# Autodesk Inventor assembly: Vex Traction Wheel 6x1
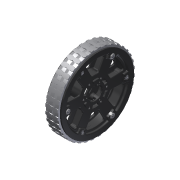
[picture p0: Inventor's stored thumbnail of the model, 180x180]
Saved by Autodesk Inventor 2013 (Build 170138000, 138)
## iProperties
Created: 2012-12-09
Part Number: Vex Traction Wheel 6x1
Document SubType Name: Assembly
Designer: Nemo
Author: Nemo
## Documents named in this file (6)
- H:\Nemo\Documents\Robotics\COTS Parts\Wheels\VexPro Traction Wheels\Vex Traction Wheel 6x1.iam
- H:\Nemo\Documents\Robotics\COTS Parts\Wheels\VexPro Traction Wheels\Components\Traction Wheel Body 6in.ipt
- H:\Nemo\Documents\Robotics\COTS Parts\Fasteners\Hex Standoff 8-32 x750.ipt
- H:\Nemo\Documents\Robotics\COTS Parts\Fasteners\8-32 locknut.ipt
- H:\Nemo\Documents\Robotics\COTS Parts\Fasteners\8-32 BHCS x1250.ipt
- H:\Nemo\Documents\Robotics\COTS Parts\Wheels\VexPro Traction Wheels\Components\6 in Traction Tire.iam
## Components (22 placed, 5 different names)
1. Traction Wheel Body 6in:1 — Mate:1, Flush:1, Mate:2, Angle:1, Insert:1, Insert:2, Angle:2, Insert:3, Mate:5, Mate:8
2. Traction Wheel Body 6in:2 — Mate:3, Mate:4, Mate:5, Insert:4, Angle:3, Insert:5
3. 6 in Traction Tire:1 [sub-assembly] — Mate:6, Mate:7, Mate:8, Mate:11
4. 6 in Traction Tire:2 [sub-assembly] — Mate:9, Mate:10, Mate:11
5. Hex Standoff 8-32 x750:1 — Angle:1, Insert:1
6. Hex Standoff 8-32 x750:2
7. Hex Standoff 8-32 x750:3
8. Hex Standoff 8-32 x750:4
9. Hex Standoff 8-32 x750:5
10. Hex Standoff 8-32 x750:6
11. 8-32 BHCS x1250:2 — Insert:4
12. 8-32 locknut:2 — Angle:3, Insert:5
13. 8-32 BHCS x1250:1 — Insert:3
14. 8-32 locknut:1 — Insert:2, Angle:2
15. 8-32 BHCS x1250:3
16. 8-32 locknut:3
17. 8-32 BHCS x1250:4
18. 8-32 locknut:4
19. 8-32 BHCS x1250:5
20. 8-32 locknut:5
21. 8-32 BHCS x1250:6
22. 8-32 locknut:6
## Component patterns: (6 elements, first: Hex Standoff 8-32 x750:1), (3 elements, first: 8-32 BHCS x1250:2 + 8-32 locknut:2 + 8-32 BHCS x1250:1 + 8-32 locknut:1)
## Relationships (20: Mate 11, Insert 5, Angle 3, Flush 1)
- Mate:1: Traction Wheel Body 6in:1
- Flush:1: Traction Wheel Body 6in:1
- Mate:2: Traction Wheel Body 6in:1
- Angle:1 (0 deg): Traction Wheel Body 6in:1 ↔ Hex Standoff 8-32 x750:1
- Insert:1: Traction Wheel Body 6in:1 ↔ Hex Standoff 8-32 x750:1
- Insert:2: Traction Wheel Body 6in:1 ↔ 8-32 locknut:1
- Angle:2 (0 deg): Traction Wheel Body 6in:1 ↔ 8-32 locknut:1
- Insert:3: Traction Wheel Body 6in:1 ↔ 8-32 BHCS x1250:1
- Mate:3: Traction Wheel Body 6in:2
- Mate:4: Traction Wheel Body 6in:2
- Mate:5: Traction Wheel Body 6in:1 ↔ Traction Wheel Body 6in:2
- Insert:4: Traction Wheel Body 6in:2 ↔ 8-32 BHCS x1250:2
- Angle:3 (0 deg): Traction Wheel Body 6in:2 ↔ 8-32 locknut:2
- Insert:5: Traction Wheel Body 6in:2 ↔ 8-32 locknut:2
- Mate:6: 6 in Traction Tire:1
- Mate:7: 6 in Traction Tire:1
- Mate:8: Traction Wheel Body 6in:1 ↔ 6 in Traction Tire:1
- Mate:9: 6 in Traction Tire:2
- Mate:10: 6 in Traction Tire:2
- Mate:11: 6 in Traction Tire:1 ↔ 6 in Traction Tire:2
